# Autodesk Inventor assembly: intakecenterer
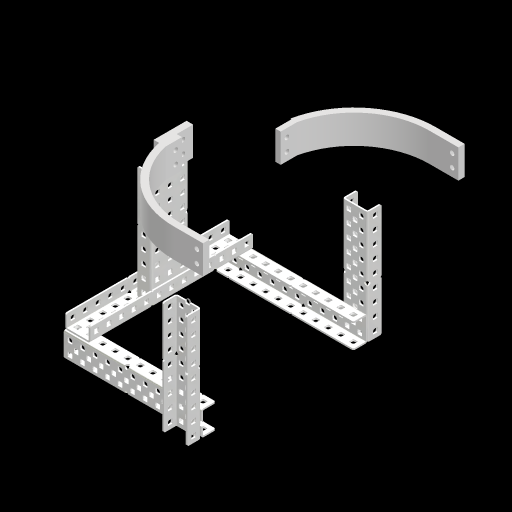
[picture p0: Inventor's stored thumbnail of the model, 512x512]
Saved by Autodesk Inventor 2024.1 (Build 281209000, 209)
## iProperties
Created: 2025-05-14
Part Number: intakecenterer
Document SubType Name: Assembly
Designer: Teddy
Author: Teddy
## Documents named in this file (6)
- C:\Users\Teddy\OneDrive\Desktop\VEX-CAD-Inventor-1.4.0\pushBack\PushBackBot2\intakecenterer.iam
- C:\Users\Teddy\OneDrive\Desktop\VEX-CAD-Inventor-1.4.0\Structure\C Channel\Aluminum 1x2x1\Alu C 1x2x1x9.ipt
- C:\Users\Teddy\OneDrive\Desktop\VEX-CAD-Inventor-1.4.0\Structure\C Channel\Aluminum 1x2x1\Alu C 1x2x1x13.ipt
- C:\Users\Teddy\OneDrive\Desktop\VEX-CAD-Inventor-1.4.0\Structure\C Channel\Aluminum 1x3x1\Alu C 1x3x1x9.ipt
- C:\Users\Teddy\OneDrive\Desktop\VEX-CAD-Inventor-1.4.0\Structure\C Channel\Aluminum 1x2x1\Alu C 1x2x1x11.ipt
- C:\Users\Teddy\OneDrive\Desktop\VEX-CAD-Inventor-1.4.0\pushBack\PushBackBot2\intakeConstraint.ipt
## Components (7 placed, 5 different names)
1. Alu C 1x2x1x9:1 — Insert:9, Insert:10
2. Alu C 1x2x1x9:2 — Insert:7, Insert:8
3. Alu C 1x2x1x13:1 — Insert:1, Insert:2, Insert:3, Insert:4, Insert:5, Insert:6
4. Alu C 1x3x1x9:1 — Insert:1, Insert:2, Flush:1, Flush:2
5. Alu C 1x2x1x11:1 — Insert:5, Insert:6, Insert:7, Insert:8
6. Alu C 1x2x1x11:2 — Insert:3, Insert:4, Insert:9, Insert:10
7. intakeConstraint:1 — Flush:1, Flush:2
## Relationships (12: Insert 10, Flush 2)
- Insert:1: Alu C 1x2x1x13:1 ↔ Alu C 1x3x1x9:1
- Insert:2: Alu C 1x2x1x13:1 ↔ Alu C 1x3x1x9:1
- Insert:3: Alu C 1x2x1x13:1 ↔ Alu C 1x2x1x11:2
- Insert:4: Alu C 1x2x1x13:1 ↔ Alu C 1x2x1x11:2
- Insert:5: Alu C 1x2x1x13:1 ↔ Alu C 1x2x1x11:1
- Insert:6: Alu C 1x2x1x13:1 ↔ Alu C 1x2x1x11:1
- Insert:7: Alu C 1x2x1x9:2 ↔ Alu C 1x2x1x11:1
- Insert:8: Alu C 1x2x1x9:2 ↔ Alu C 1x2x1x11:1
- Insert:9: Alu C 1x2x1x9:1 ↔ Alu C 1x2x1x11:2
- Insert:10: Alu C 1x2x1x9:1 ↔ Alu C 1x2x1x11:2
- Flush:1: Alu C 1x3x1x9:1 ↔ intakeConstraint:1
- Flush:2: Alu C 1x3x1x9:1 ↔ intakeConstraint:1
